# Autodesk Inventor assembly: motor_sb
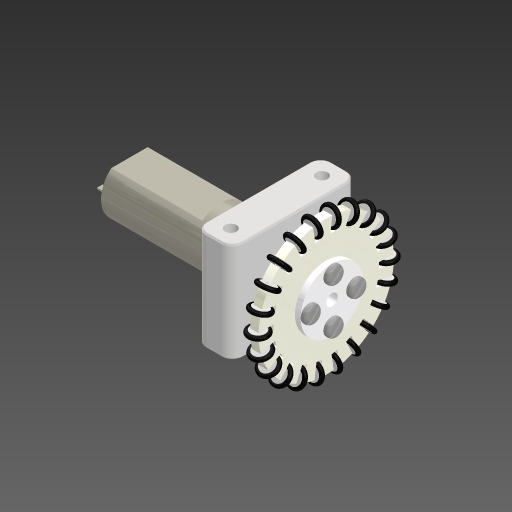
[picture p0: Inventor's stored thumbnail of the model, 512x512]
Saved by Autodesk Inventor 2023 (Build 270158000, 158)
## iProperties
Created: 2025-09-23
Part Number: motor_sb
Document SubType Name: Assembly
Designer: daa
Author: daa
## Documents named in this file (4)
- C:\Users\daa\Documents\DASH_V2\omni_platforma\motor_sb.iam
- C:\Users\daa\Documents\DASH_V2\omni_platforma\fastenin_motor.ipt
- C:\Users\daa\Documents\DASH_V2\omni_platforma\motor20.ipt
- C:\Users\daa\Documents\DASH_V2\omni_platforma\Wheel.iam
## Components (3 placed, 3 different names)
1. fastenin_motor:1 — С поворотом:1
2. motor20:1 — С поворотом:1, С поворотом:2
3. Wheel:1 [sub-assembly] — С поворотом:2
## Relationships (2: RevoluteJoint 2)
- С поворотом:1 [RevoluteJoint] (-6 mm): fastenin_motor:1 ↔ motor20:1
- С поворотом:2 [RevoluteJoint] (-5 mm): motor20:1 ↔ Wheel:1
